# Autodesk Inventor assembly: MGN15 Linear Rail 1000mm - 4040 Assembly
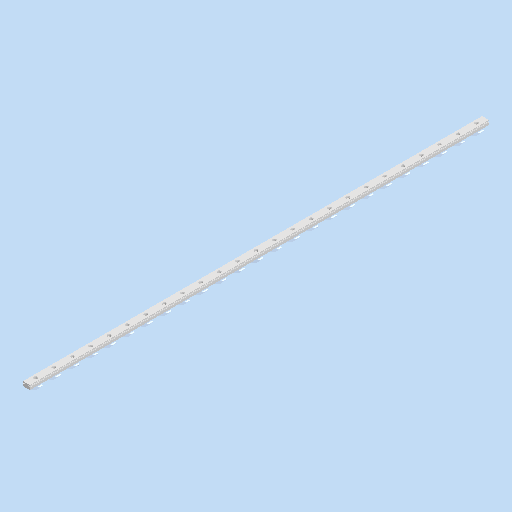
[picture p0: Inventor's stored thumbnail of the model, 512x512]
Saved by Autodesk Inventor 2023.2 (Build 272271000, 271)
## iProperties
Created: 2023-11-23
Part Number: MGN15 Linear Rail 1000mm - 4040 Assembly
Document SubType Name: Assembly
Designer: Nils Bade
Author: Nils Bade
## Documents named in this file (4)
- C:\Users\nilsb\Documents\Inventor\Projektarbeit-Bade\RatRig_modified\MGN15 Linear Rail 1000mm - 4040 Assembly.iam
- C:\Users\nilsb\Documents\Inventor\Projektarbeit-Bade\RatRig_modified\MGN15 Linear Rail 1000mm.ipt
- C:\Users\nilsb\Documents\Inventor\Projektarbeit-Bade\Schrauben\Cap Head Screw M3x12 v2.ipt
- C:\Users\nilsb\Documents\Inventor\Projektarbeit-Bade\ITEM\item_Nutenstein 8 - M3_37359.ipt
## Components (51 placed, 3 different names)
1. MGN15 Linear Rail 1000mm:1 — Passend:1, Passend:2, Passend:5
2. item_Nutenstein 8 - M3_37359:1 — Passend:3, Passend:4, Passend:5
3. Cap Head Screw M3x12 v2:1 — Passend:1, Passend:2, Passend:4
4. item_Nutenstein 8 - M3_37359:2
5. Cap Head Screw M3x12 v2:2
6. item_Nutenstein 8 - M3_37359:3
7. Cap Head Screw M3x12 v2:3
8. item_Nutenstein 8 - M3_37359:4
9. Cap Head Screw M3x12 v2:4
10. item_Nutenstein 8 - M3_37359:5
11. Cap Head Screw M3x12 v2:5
12. item_Nutenstein 8 - M3_37359:6
13. Cap Head Screw M3x12 v2:6
14. item_Nutenstein 8 - M3_37359:7
15. Cap Head Screw M3x12 v2:7
16. item_Nutenstein 8 - M3_37359:8
17. Cap Head Screw M3x12 v2:8
18. item_Nutenstein 8 - M3_37359:9
19. Cap Head Screw M3x12 v2:9
20. item_Nutenstein 8 - M3_37359:10
21. Cap Head Screw M3x12 v2:10
22. item_Nutenstein 8 - M3_37359:11
23. Cap Head Screw M3x12 v2:11
24. item_Nutenstein 8 - M3_37359:12
25. Cap Head Screw M3x12 v2:12
26. item_Nutenstein 8 - M3_37359:13
27. Cap Head Screw M3x12 v2:13
28. item_Nutenstein 8 - M3_37359:14
29. Cap Head Screw M3x12 v2:14
30. item_Nutenstein 8 - M3_37359:15
31. Cap Head Screw M3x12 v2:15
32. item_Nutenstein 8 - M3_37359:16
33. Cap Head Screw M3x12 v2:16
34. item_Nutenstein 8 - M3_37359:17
35. Cap Head Screw M3x12 v2:17
36. item_Nutenstein 8 - M3_37359:18
37. Cap Head Screw M3x12 v2:18
38. item_Nutenstein 8 - M3_37359:19
39. Cap Head Screw M3x12 v2:19
40. item_Nutenstein 8 - M3_37359:20
41. Cap Head Screw M3x12 v2:20
42. item_Nutenstein 8 - M3_37359:21
43. Cap Head Screw M3x12 v2:21
44. item_Nutenstein 8 - M3_37359:22
45. Cap Head Screw M3x12 v2:22
46. item_Nutenstein 8 - M3_37359:23
47. Cap Head Screw M3x12 v2:23
48. item_Nutenstein 8 - M3_37359:24
49. Cap Head Screw M3x12 v2:24
50. item_Nutenstein 8 - M3_37359:25
51. Cap Head Screw M3x12 v2:25
## Component patterns: (25 elements, first: item_Nutenstein 8 - M3_37359:1 + Cap Head Screw M3x12 v2:1)
## Relationships (5: Mate 5)
- Passend:1 [Mate]: MGN15 Linear Rail 1000mm:1 ↔ Cap Head Screw M3x12 v2:1
- Passend:2 [Mate]: MGN15 Linear Rail 1000mm:1 ↔ Cap Head Screw M3x12 v2:1
- Passend:3 [Mate]: item_Nutenstein 8 - M3_37359:1
- Passend:4 [Mate]: item_Nutenstein 8 - M3_37359:1 ↔ Cap Head Screw M3x12 v2:1
- Passend:5 [Mate] (5.5 mm): MGN15 Linear Rail 1000mm:1 ↔ item_Nutenstein 8 - M3_37359:1
